# Autodesk Inventor assembly: Ensamble_Base
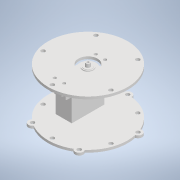
[picture p0: Inventor's stored thumbnail of the model, 180x180]
Saved by Autodesk Inventor 2022 (Build 260153000, 153)
## iProperties
Created: 2021-09-23
Part Number: Ensamble_Base
Document SubType Name: Assembly
Designer: Administrador
Author: Administrador
## Documents named in this file (4)
- C:\Users\Administrador\Desktop\Octavo Semestre\Robótica Industrial\Robot\Links\Link_Base.iam
- C:\Users\Administrador\Desktop\Octavo Semestre\Robótica Industrial\Robot\Cuerpo\PartesCuerpo\Base_Suelo.ipt
- C:\Users\Administrador\Desktop\Octavo Semestre\Robótica Industrial\Robot\Cuerpo\PartesCuerpo\Base2.ipt
- C:\Users\Administrador\Desktop\Octavo Semestre\Robótica Industrial\Robot\Cuerpo\PartesCuerpo\Motor Mg995.ipt
## Components (3 placed, 3 different names)
1. Base_Suelo:1
2. Base2:1
3. Motor Mg995:1
## Relationships (6: Mate 5, WeldJoint 1)
- [WeldJoint] (54 mm): Base_Suelo:1 ↔ Base2:1
- [Mate]: Base2:1 ↔ Motor Mg995:1
- [Mate]: Base2:1 ↔ Motor Mg995:1
- [Mate]: Base2:1 ↔ Motor Mg995:1
- [Mate]: Base2:1 ↔ Motor Mg995:1
- [Mate]: Base2:1 ↔ Motor Mg995:1
